# Autodesk Inventor assembly: Assemble
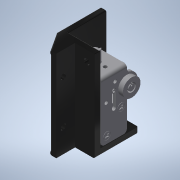
[picture p0: Inventor's stored thumbnail of the model, 180x180]
Saved by Autodesk Inventor 2021 (Build 250183000, 183)
## iProperties
Created: 2019-07-20
Part Number: Assemble
Material: 一般
Document SubType Name: Assembly
Designer: gisen
Author: gisen
## Documents named in this file (3)
- D:\GitProjects\CAD-Data\Devices\SolenoidLatch\SolenoidLatchAssembly.iam
- D:\GitProjects\CAD-Data\Devices\SolenoidLatch\SolenoidLatch.iam
- D:\GitProjects\CAD-Data\Devices\SolenoidLatch\SolenoidLatchMount.ipt
## Components (2 placed, 2 different names)
1. SolenoidLatch:1 [sub-assembly] — フラッシュ:1
2. SolenoidLatchMount:1 — フラッシュ:1, メイト:1, メイト:2
## Relationships (3: Mate 2, Flush 1)
- フラッシュ:1 [Flush]: SolenoidLatch:1 ↔ SolenoidLatchMount:1
- メイト:1 [Mate]: SolenoidLatchMount:1
- メイト:2 [Mate]: SolenoidLatchMount:1
